# Autodesk Inventor assembly: legg_assembly
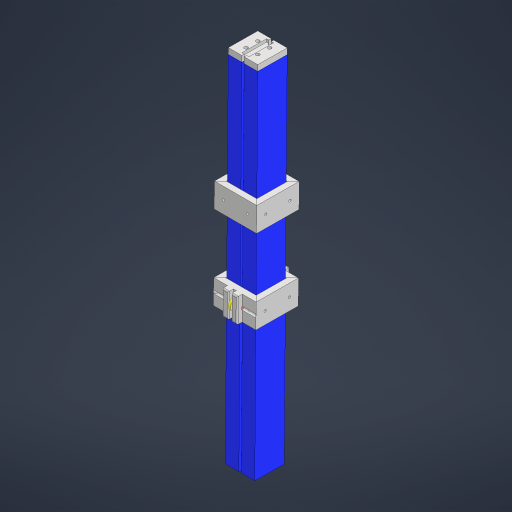
[picture p0: Inventor's stored thumbnail of the model, 512x512]
Saved by Autodesk Inventor 2024 (Build 280153000, 153)
## iProperties
Created: 2023-05-23
Part Number: legg_assembly
Document SubType Name: Assembly
Designer: aasmu
Author: aasmu
## Documents named in this file (5)
- C:\Users\aasmu\Documents\standing_desk\legg_assembly.iam
- C:\Users\aasmu\Documents\standing_desk\1_inner_leg.ipt
- C:\Users\aasmu\Documents\standing_desk\2_inner_leg_top_plate.ipt
- C:\Users\aasmu\Documents\standing_desk\inner_glide_carriage_assembly.iam
- C:\Users\aasmu\Documents\standing_desk\inner_glide_carriage_with_roller_assembly.iam
## Components (4 placed, 4 different names)
1. 1_inner_leg:1 — Rigid:1, Mate:1, Mate:2, Mate:3, Mate:4
2. 2_inner_leg_top_plate:1 — Rigid:1
3. inner_glide_carriage_assembly:1 [sub-assembly] — Mate:1, Mate:2
4. inner_glide_carriage_with_roller_assembly:1 [sub-assembly] — Mate:3, Mate:4
## Relationships (5: Mate 4, WeldJoint 1)
- Rigid:1 [WeldJoint]: 1_inner_leg:1 ↔ 2_inner_leg_top_plate:1
- Mate:1: 1_inner_leg:1 ↔ inner_glide_carriage_assembly:1
- Mate:2: 1_inner_leg:1 ↔ inner_glide_carriage_assembly:1
- Mate:3: 1_inner_leg:1 ↔ inner_glide_carriage_with_roller_assembly:1
- Mate:4: 1_inner_leg:1 ↔ inner_glide_carriage_with_roller_assembly:1
